# Autodesk Inventor assembly: LiftFull
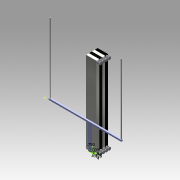
[picture p0: Inventor's stored thumbnail of the model, 180x180]
Saved by Autodesk Inventor 2016 (Build 200138000, 138)
## iProperties
Created: 2017-02-22
Part Number: LiftFull
Document SubType Name: Assembly
Designer: Delta
Author: Delta
## Documents named in this file (3)
- C:\Robotics\CAD\2016-17_CAD\LiftFull.iam
- C:\Robotics\CAD\2016-17_CAD\Lift.iam
- C:\Robotics\CAD\2016-17_CAD\HingeMK3.iam
## Components (2 placed, 2 different names)
1. Lift:1 [sub-assembly] — Mate:1, Flush:1, Flush:2
2. HingeMK3:1 [sub-assembly] — Mate:1, Flush:1, Flush:2
## Relationships (3: Flush 2, Mate 1)
- Mate:1: Lift:1 ↔ HingeMK3:1
- Flush:1: Lift:1 ↔ HingeMK3:1
- Flush:2 (13.97 mm): Lift:1 ↔ HingeMK3:1
